# Autodesk Inventor assembly: 2018 zentai assembly
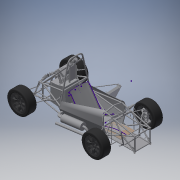
[picture p0: Inventor's stored thumbnail of the model, 180x180]
Saved by Autodesk Inventor 2018 (Build 220112000, 112)
## iProperties
Company: none
Created: 2018-03-10
Part Number: 2018 zentai assembly
Material: 一般
Description: CATIA V5 STEP Exchange
Document SubType Name: Assembly
Designer: ku_sk
Authority: none
Title: Z:\各班フォルダ\2018\ボディ\カウル\Aero\KS-15\body\2018 zentai assembly for kuwano.stp
Author: none
## Documents named in this file (27)
- D:\Users\ku_sk\Documents\Inventor\Aero\KS-15\body\2018 zentai assembly.iam
- D:\Users\ku_sk\Documents\Inventor\Aero\KS-15\body\parts\karikuni12a.ipt
- D:\Users\ku_sk\Documents\Inventor\Aero\KS-15\body\parts\Bracket.iam
- D:\Users\ku_sk\Documents\Inventor\Aero\KS-15\body\parts\2018 Exhaust assembly.iam
- D:\Users\ku_sk\Documents\Inventor\Aero\KS-15\body\parts\seat for human 2018.ipt
- D:\Users\ku_sk\Documents\Inventor\Aero\KS-15\body\parts\shifter.iam
- D:\Users\ku_sk\Documents\Inventor\Aero\KS-15\body\parts\CL_engine_to_rad.ipt
- D:\Users\ku_sk\Documents\Inventor\Aero\KS-15\body\parts\radiator 2018.ipt
- D:\Users\ku_sk\Documents\Inventor\Aero\KS-15\body\parts\2018 Intake.iam
- D:\Users\ku_sk\Documents\Inventor\Aero\KS-15\body\parts\radiator stay Lower.ipt
- D:\Users\ku_sk\Documents\Inventor\Aero\KS-15\body\parts\AssyTsutsui2018A.iam
- D:\Users\ku_sk\Documents\Inventor\Aero\KS-15\body\parts\rad stay rod.ipt
- D:\Users\ku_sk\Documents\Inventor\Aero\KS-15\body\parts\radiator stay SIR.ipt
- D:\Users\ku_sk\Documents\Inventor\Aero\KS-15\body\parts\F-Upright2018.iam
- D:\Users\ku_sk\Documents\Inventor\Aero\KS-15\body\parts\F-Upright2018-symmetory.iam
- D:\Users\ku_sk\Documents\Inventor\Aero\KS-15\body\parts\R-Upright2018-symmetory.iam
- D:\Users\ku_sk\Documents\Inventor\Aero\KS-15\body\parts\R-Upright2018.iam
- D:\Users\ku_sk\Documents\Inventor\Aero\KS-15\body\parts\SidePanel_Upper.ipt
- D:\Users\ku_sk\Documents\Inventor\Aero\KS-15\body\parts\chain cover stay upper.ipt
- D:\Users\ku_sk\Documents\Inventor\Aero\KS-15\body\parts\chaincover stay lower.ipt
- D:\Users\ku_sk\Documents\Inventor\Aero\KS-15\body\parts\AcceleratorWireStay.ipt
- D:\Users\ku_sk\Documents\Inventor\Aero\KS-15\body\parts\Frontunderpanel.ipt
- D:\Users\ku_sk\Documents\Inventor\Aero\KS-15\body\parts\Frontnose braket.ipt
- D:\Users\ku_sk\Documents\Inventor\Aero\KS-15\body\parts\simplicity engine.ipt
- D:\Users\ku_sk\Documents\Inventor\Aero\KS-15\Fr.wing\parts\stay\Bracket.ipt
- D:\Users\ku_sk\Documents\Inventor\Aero\KS-15\Fr.wing\parts\stay\Bracket1.ipt
- D:\Users\ku_sk\Documents\Inventor\Aero\KS-15\body\parts\2015Wheel watanabe.ipt
## Components (29 placed, 26 different names)
1. karikuni12a.1 — メイト:1, メイト:2
2. Bracket.1 [sub-assembly]
3. 2018 Exhaust assembly.1 [sub-assembly]
4. seat for human 2018.1
5. shifter.1 [sub-assembly]
6. Part2.1
7. radiator 2018.2
8. 2018 Intake.1 [sub-assembly]
9. radiator stay Lower.2
10. AssyTsutsui2018A.1 [sub-assembly]
11. Part2.3
12. radiator stay SIR.1
13. F-Upright2018.1 [sub-assembly] — フラッシュ:1, メイト:3, フラッシュ:2, メイト:9
14. F-Upright2018-symmetory.1 [sub-assembly] — フラッシュ:1, メイト:3, フラッシュ:2, メイト:10
15. R-Upright2018-symmetory.2 [sub-assembly] — メイト:4, フラッシュ:3, フラッシュ:4, メイト:5, メイト:6
16. R-Upright2018.2 [sub-assembly] — メイト:4, フラッシュ:3, フラッシュ:4, メイト:7, メイト:8
17. SidePanel_Upper.1
18. chain cover stay upper
19. chaincover stay lower
20. AcceleratorWireStay.1
21. Frontunderpanel.1
22. Frontnose braket.1
23. simplicity engine.1
24. Bracket:2 — メイト:1, メイト:2
25. Bracket1:1
26. 2015Wheel watanabe:1 — メイト:5, メイト:6, フラッシュ:6
27. 2015Wheel watanabe:2 — メイト:7, メイト:8, フラッシュ:5
28. 2015Wheel watanabe:3 — フラッシュ:5, メイト:9
29. 2015Wheel watanabe:4 — メイト:10, フラッシュ:6
## Relationships (16: Mate 10, Flush 6)
- メイト:1 [Mate]: karikuni12a.1 ↔ Bracket:2
- メイト:2 [Mate]: karikuni12a.1 ↔ Bracket:2
- フラッシュ:1 [Flush]: F-Upright2018.1 ↔ F-Upright2018-symmetory.1
- メイト:3 [Mate] (1057.6 mm): F-Upright2018.1 ↔ F-Upright2018-symmetory.1
- フラッシュ:2 [Flush]: F-Upright2018.1 ↔ F-Upright2018-symmetory.1
- メイト:4 [Mate] (1064 mm): R-Upright2018-symmetory.2 ↔ R-Upright2018.2
- フラッシュ:3 [Flush]: R-Upright2018-symmetory.2 ↔ R-Upright2018.2
- フラッシュ:4 [Flush]: R-Upright2018-symmetory.2 ↔ R-Upright2018.2
- メイト:5 [Mate] (49 mm): R-Upright2018-symmetory.2 ↔ 2015Wheel watanabe:1
- メイト:6 [Mate]: R-Upright2018-symmetory.2 ↔ 2015Wheel watanabe:1
- メイト:7 [Mate] (49 mm): R-Upright2018.2 ↔ 2015Wheel watanabe:2
- メイト:8 [Mate]: R-Upright2018.2 ↔ 2015Wheel watanabe:2
- フラッシュ:5 [Flush]: 2015Wheel watanabe:2 ↔ 2015Wheel watanabe:3
- メイト:9 [Mate]: F-Upright2018.1 ↔ 2015Wheel watanabe:3
- メイト:10 [Mate]: F-Upright2018-symmetory.1 ↔ 2015Wheel watanabe:4
- フラッシュ:6 [Flush]: 2015Wheel watanabe:1 ↔ 2015Wheel watanabe:4
